# Autodesk Inventor assembly: robot1
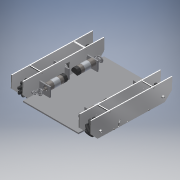
[picture p0: Inventor's stored thumbnail of the model, 180x180]
Saved by Autodesk Inventor 2019 (Build 230136000, 136)
## iProperties
Created: 2020-10-03
Part Number: robot1
Document SubType Name: Assembly
Designer: User
Author: User
## Documents named in this file (8)
- C:\Robotics\CAD\2020-21-CAD\main robot\robot1.iam
- C:\Robotics\CAD\2020-21-CAD\main robot\main plate.ipt
- C:\Robotics\CAD\2020-21-CAD\Drivetrain\drive train right.iam
- C:\Robotics\CAD\2020-21-CAD\Drivetrain\drive train left.iam
- C:\Robotics\CAD\2020-21-CAD\Drivetrain\third odomitry wheel.ipt
- C:\Robotics\CAD\COTSParts\Rev\REV-11-1271.STEP encoders.ipt
- C:\Robotics\CAD\COTSParts\andymark\am-3902 am-3903 2in Omni 14mm Hex.ipt
- C:\Robotics\CAD\2020-21-CAD\Shooter\Shooter Assembly.iam
## Components (7 placed, 7 different names)
1. main plate:1 — Mate:3, Mate:4, Mate:20, Mate:23, Mate:25, Mate:28, Flush:1
2. drive train right:1 [sub-assembly] — Mate:3, Mate:22, Mate:24, Mate:25, Mate:27
3. drive train left:1 [sub-assembly] — Mate:4, Mate:28, Flush:1
4. third odomitry wheel:1 — Mate:18, Angle:1, Mate:20, Mate:21, Mate:22, Mate:27
5. REV-11-1271.STEP encoders:1 — Mate:14, Mate:15, Mate:18, Angle:1, Mate:21
6. am-3902 am-3903 2in Omni 14mm Hex:1 — Mate:14, Mate:15
7. Shooter Assembly:1 [sub-assembly] — Mate:23, Mate:24
## Relationships (15: Mate 13, Angle 1, Flush 1)
- Mate:3: main plate:1 ↔ drive train right:1
- Mate:4: main plate:1 ↔ drive train left:1
- Mate:14: REV-11-1271.STEP encoders:1 ↔ am-3902 am-3903 2in Omni 14mm Hex:1
- Mate:15: REV-11-1271.STEP encoders:1 ↔ am-3902 am-3903 2in Omni 14mm Hex:1
- Mate:18: third odomitry wheel:1 ↔ REV-11-1271.STEP encoders:1
- Angle:1 (15 deg): third odomitry wheel:1 ↔ REV-11-1271.STEP encoders:1
- Mate:20: main plate:1 ↔ third odomitry wheel:1
- Mate:21: third odomitry wheel:1 ↔ REV-11-1271.STEP encoders:1
- Mate:22: drive train right:1 ↔ third odomitry wheel:1
- Mate:23: main plate:1 ↔ Shooter Assembly:1
- Mate:24: drive train right:1 ↔ Shooter Assembly:1
- Mate:25: main plate:1 ↔ drive train right:1
- Mate:27: drive train right:1 ↔ third odomitry wheel:1
- Mate:28: main plate:1 ↔ drive train left:1
- Flush:1: main plate:1 ↔ drive train left:1
